# Autodesk Inventor assembly: LinearActuator400mm
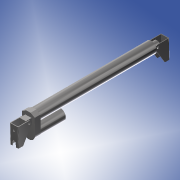
[picture p0: Inventor's stored thumbnail of the model, 180x180]
Saved by Autodesk Inventor 2017 SP1 (Build 210196100, 196)
## iProperties
Created: 2017-07-19
Part Number: LinearActuator400mm
Document SubType Name: Assembly
Designer: zallen
Author: zallen
## Documents named in this file (3)
- C:\Users\Zach\Documents\GitHub\cr-laundry-robot\lib\Linear Actuator 300mm\LinearActuator300mm.iam
- C:\Users\Zach\Documents\GitHub\cr-laundry-robot\lib\Linear Actuator 300mm\LinearActuator300mm.ipt
- C:\Users\Zach\Documents\GitHub\cr-laundry-robot\lib\Linear Actuator 300mm\Mount.ipt
## Components (3 placed, 2 different names)
1. LinearActuator300mm:1 — Mate:1, Mate:4, Mate:5, Mate:7, Angle:1, Tangent:1, Mate:8
2. Mount:1 — Mate:1, Mate:3, Mate:8, Mate:9
3. Mount:2 — Mate:7, Angle:1, Tangent:1
## Relationships (9: Mate 7, Angle 1, Tangent 1)
- Mate:1: LinearActuator300mm:1 ↔ Mount:1
- Mate:3: Mount:1
- Mate:4: LinearActuator300mm:1
- Mate:5: LinearActuator300mm:1
- Mate:7: LinearActuator300mm:1 ↔ Mount:2
- Angle:1 (0 deg): LinearActuator300mm:1 ↔ Mount:2
- Tangent:1: LinearActuator300mm:1 ↔ Mount:2
- Mate:8: LinearActuator300mm:1 ↔ Mount:1
- Mate:9: Mount:1
